# Autodesk Inventor assembly: Gantry2
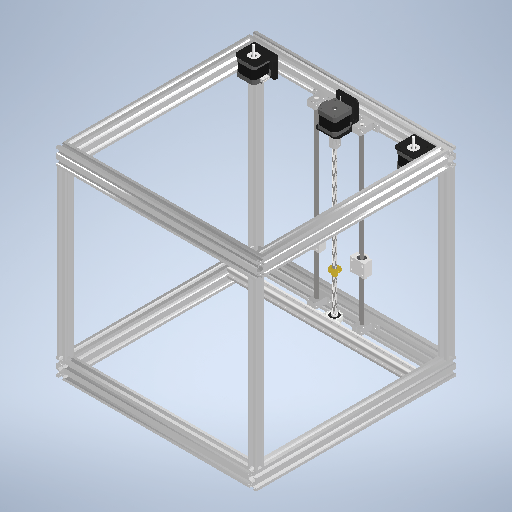
[picture p0: Inventor's stored thumbnail of the model, 512x512]
Saved by Autodesk Inventor 2025.2 (Build 292293000, 293)
## iProperties
Created: 2025-07-13
Part Number: Gantry2
Document SubType Name: Assembly
Designer: Simon
Author: Simon
## Documents named in this file (14)
- C:\Users\Simon\Projects\Hydrogel-3D-Printer\Hardware\Bioprinter Machine Design\Gantry Concept 2\Gantry2.iam
- C:\Users\Simon\Projects\Hydrogel-3D-Printer\Hardware\Bioprinter Machine Design\Gantry Concept 2\2040_AluminimProfile_410.ipt
- C:\Users\Simon\Projects\Hydrogel-3D-Printer\Hardware\Bioprinter Machine Design\Gantry Concept 2\2040_AluminimProfile_450.ipt
- C:\Users\Simon\Projects\Hydrogel-3D-Printer\Hardware\Bioprinter Machine Design\Gantry Concept 2\2020_AluminiumProfile_370.ipt
- C:\Users\Simon\Projects\Hydrogel-3D-Printer\Hardware\Bioprinter Machine Design\PartsFolder\Stepper_17HS4401.ipt
- C:\Users\Simon\Projects\Hydrogel-3D-Printer\Hardware\Bioprinter Machine Design\PartsFolder\bracket nema 17.ipt
- C:\Users\Simon\Projects\Hydrogel-3D-Printer\Hardware\Bioprinter Machine Design\PartsFolder\Pillow Block Bearing 2\KP08_2.iam
- C:\Users\Simon\Projects\Hydrogel-3D-Printer\Hardware\Bioprinter Machine Design\Gantry Concept 2\2020_AluminiumProfile_410.ipt
- C:\Users\Simon\Projects\Hydrogel-3D-Printer\Hardware\Bioprinter Machine Design\Gantry Concept 2\TR8x8-4_LeadScrew_350mm.ipt
- C:\Users\Simon\Projects\Hydrogel-3D-Printer\Hardware\Bioprinter Machine Design\PartsFolder\TR8x8-4_Nut.ipt
- C:\Users\Simon\Projects\Hydrogel-3D-Printer\Hardware\Bioprinter Machine Design\PartsFolder\SK8_LinearShaftSupport.ipt
- C:\Users\Simon\Projects\Hydrogel-3D-Printer\Hardware\Bioprinter Machine Design\PartsFolder\Flexible Coupling 5,8.ipt
- C:\Users\Simon\Projects\Hydrogel-3D-Printer\Hardware\Bioprinter Machine Design\Gantry Concept 2\SteelShaft_404mm.ipt
- C:\Users\Simon\Projects\Hydrogel-3D-Printer\Hardware\Bioprinter Machine Design\PartsFolder\SC8UU\SC8UU.iam
## Components (31 placed, 13 different names)
1. 2040_AluminimProfile_410:1 — Mate:16, Flush:16, Flush:17, Mate:37
2. 2040_AluminimProfile_450:1 — Mate:15, Flush:14, Flush:15, Flush:16, Mate:17, Flush:18, Flush:19, Flush:20, Mate:20, Mate:28, Angle:3, Mate:35, Mate:36, Flush:36, Flush:37
3. 2040_AluminimProfile_410:2 — Mate:6, Mate:7, Flush:3, Angle:2
4. 2040_AluminimProfile_450:2 — Mate:2, Flush:1, Mate:4, Mate:7, Flush:3, Mate:8, Mate:10, Flush:4, Flush:5, Mate:11, Flush:6, Flush:7, Mate:22, Flush:21
5. 2040_AluminimProfile_410:3 — Mate:3, Mate:4, Mate:5, Flush:2
6. 2040_AluminimProfile_450:3 — Mate:1, Flush:1, Mate:5, Flush:2, Mate:9, Mate:12, Mate:13, Flush:8, Flush:9, Flush:10, Flush:11, Mate:29
7. 2040_AluminimProfile_410:4 — Mate:17, Flush:18, Flush:19, Mate:30, Mate:38
8. 2040_AluminimProfile_450:4 — Mate:14, Flush:12, Flush:13, Mate:16, Flush:17
9. 2020_AluminiumProfile_370:1 — Mate:13, Flush:10, Flush:11, Mate:14, Flush:12, Flush:13
10. 2020_AluminiumProfile_370:2 — Mate:12, Flush:8, Flush:9, Mate:15, Flush:14, Flush:15
11. 2020_AluminiumProfile_370:3 — Mate:11, Flush:6, Flush:7
12. 2020_AluminiumProfile_370:4 — Mate:10, Flush:4, Flush:5
13. Stepper_17HS4401:1 — Mate:39, Mate:41, Angle:4
14. Stepper_17HS4401:2 — Mate:40, Mate:42, Angle:5
15. Stepper_17HS4401:3 — Mate:18, Mate:19, Angle:1, Mate:21, Mate:25, Flush:23
16. bracket nema 17:1 — Mate:36, Flush:37, Mate:38, Mate:40, Mate:42, Angle:5
17. bracket nema 17:2 — Mate:18, Mate:19, Angle:1, Mate:20, Flush:20, Mate:31, Mate:32
18. bracket nema 17:3 — Mate:35, Flush:36, Mate:37, Mate:39, Mate:41, Angle:4
19. KP08_2:1 [sub-assembly] — Mate:21, Mate:23, Flush:22, Mate:24, Flush:24
20. 2020_AluminiumProfile_410:1 — Mate:22, Flush:21, Mate:23, Flush:22, Mate:24
21. TR8x8-4_LeadScrew_350mm:1 — Mate:25, Mate:26, Mate:27, Flush:24
22. TR8x8-4_Nut:1 — Mate:26
23. SK8_LinearShaftSupport:1 — Flush:27, Flush:31, Flush:32
24. SK8_LinearShaftSupport:2 — Flush:26, Flush:27, Flush:30, Flush:33
25. SK8_LinearShaftSupport:3 — Flush:25, Mate:28, Flush:28, Flush:32, Mate:31, Mate:33, Flush:34
26. SK8_LinearShaftSupport:4 — Flush:25, Flush:26, Flush:29, Flush:33, Mate:32, Mate:34, Flush:35
27. Flexible Coupling 5,8:1 — Mate:27, Flush:23
28. SteelShaft_404mm:1 — Mate:33, Flush:34, Mate:43
29. SteelShaft_404mm:2 — Mate:34, Flush:35, Mate:44
30. SC8UU:1 [sub-assembly] — Mate:43, Flush:38, Flush:39
31. SC8UU:2 [sub-assembly] — Mate:44, Flush:38, Flush:39
## Relationships (88: Mate 44, Flush 39, Angle 5)
- Mate:1: 2040_AluminimProfile_450:3
- Mate:2: 2040_AluminimProfile_450:2
- Flush:1: 2040_AluminimProfile_450:2 ↔ 2040_AluminimProfile_450:3
- Mate:3: 2040_AluminimProfile_410:3
- Mate:4: 2040_AluminimProfile_450:2 ↔ 2040_AluminimProfile_410:3
- Mate:5: 2040_AluminimProfile_410:3 ↔ 2040_AluminimProfile_450:3
- Flush:2: 2040_AluminimProfile_410:3 ↔ 2040_AluminimProfile_450:3
- Mate:6: 2040_AluminimProfile_410:2
- Mate:7: 2040_AluminimProfile_410:2 ↔ 2040_AluminimProfile_450:2
- Flush:3: 2040_AluminimProfile_410:2 ↔ 2040_AluminimProfile_450:2
- Mate:8: 2040_AluminimProfile_450:2
- Mate:9: 2040_AluminimProfile_450:3
- Mate:10: 2040_AluminimProfile_450:2 ↔ 2020_AluminiumProfile_370:4
- Flush:4: 2040_AluminimProfile_450:2 ↔ 2020_AluminiumProfile_370:4
- Flush:5: 2040_AluminimProfile_450:2 ↔ 2020_AluminiumProfile_370:4
- Mate:11: 2040_AluminimProfile_450:2 ↔ 2020_AluminiumProfile_370:3
- Mate:12: 2040_AluminimProfile_450:3 ↔ 2020_AluminiumProfile_370:2
- Mate:13: 2040_AluminimProfile_450:3 ↔ 2020_AluminiumProfile_370:1
- Flush:6: 2040_AluminimProfile_450:2 ↔ 2020_AluminiumProfile_370:3
- Flush:7: 2040_AluminimProfile_450:2 ↔ 2020_AluminiumProfile_370:3
- Flush:8: 2040_AluminimProfile_450:3 ↔ 2020_AluminiumProfile_370:2
- Flush:9: 2040_AluminimProfile_450:3 ↔ 2020_AluminiumProfile_370:2
- Flush:10: 2040_AluminimProfile_450:3 ↔ 2020_AluminiumProfile_370:1
- Flush:11: 2040_AluminimProfile_450:3 ↔ 2020_AluminiumProfile_370:1
- Mate:14: 2040_AluminimProfile_450:4 ↔ 2020_AluminiumProfile_370:1
- Flush:12: 2040_AluminimProfile_450:4 ↔ 2020_AluminiumProfile_370:1
- Flush:13: 2040_AluminimProfile_450:4 ↔ 2020_AluminiumProfile_370:1
- Mate:15: 2040_AluminimProfile_450:1 ↔ 2020_AluminiumProfile_370:2
- Flush:14: 2040_AluminimProfile_450:1 ↔ 2020_AluminiumProfile_370:2
- Flush:15: 2040_AluminimProfile_450:1 ↔ 2020_AluminiumProfile_370:2
- Mate:16: 2040_AluminimProfile_410:1 ↔ 2040_AluminimProfile_450:4
- Flush:16: 2040_AluminimProfile_410:1 ↔ 2040_AluminimProfile_450:1
- Flush:17: 2040_AluminimProfile_410:1 ↔ 2040_AluminimProfile_450:4
- Mate:17: 2040_AluminimProfile_450:1 ↔ 2040_AluminimProfile_410:4
- Flush:18: 2040_AluminimProfile_450:1 ↔ 2040_AluminimProfile_410:4
- Flush:19: 2040_AluminimProfile_450:1 ↔ 2040_AluminimProfile_410:4
- Mate:18: Stepper_17HS4401:3 ↔ bracket nema 17:2
- Mate:19: Stepper_17HS4401:3 ↔ bracket nema 17:2
- Angle:1 (0 deg): Stepper_17HS4401:3 ↔ bracket nema 17:2
- Mate:20: 2040_AluminimProfile_450:1 ↔ bracket nema 17:2
- Mate:21: Stepper_17HS4401:3 ↔ KP08_2:1
- Flush:20: 2040_AluminimProfile_450:1 ↔ bracket nema 17:2
- Mate:22: 2040_AluminimProfile_450:2 ↔ 2020_AluminiumProfile_410:1
- Flush:21: 2040_AluminimProfile_450:2 ↔ 2020_AluminiumProfile_410:1
- Mate:23: KP08_2:1 ↔ 2020_AluminiumProfile_410:1
- Flush:22: KP08_2:1 ↔ 2020_AluminiumProfile_410:1
- Mate:24: KP08_2:1 ↔ 2020_AluminiumProfile_410:1
- Mate:25: Stepper_17HS4401:3 ↔ TR8x8-4_LeadScrew_350mm:1
- Mate:26: TR8x8-4_LeadScrew_350mm:1 ↔ TR8x8-4_Nut:1
- Mate:27: TR8x8-4_LeadScrew_350mm:1 ↔ Flexible Coupling 5,8:1
- Flush:23 (5 mm): Stepper_17HS4401:3 ↔ Flexible Coupling 5,8:1
- Flush:24: KP08_2:1 ↔ TR8x8-4_LeadScrew_350mm:1
- Flush:25: SK8_LinearShaftSupport:3 ↔ SK8_LinearShaftSupport:4
- Flush:26: SK8_LinearShaftSupport:2 ↔ SK8_LinearShaftSupport:4
- Flush:27: SK8_LinearShaftSupport:1 ↔ SK8_LinearShaftSupport:2
- Mate:28: 2040_AluminimProfile_450:1 ↔ SK8_LinearShaftSupport:3
- Mate:29: 2040_AluminimProfile_450:3
- Angle:2 (0 deg): 2040_AluminimProfile_410:2
- Mate:30: 2040_AluminimProfile_410:4
- Angle:3 (0 deg): 2040_AluminimProfile_450:1
- Flush:28: SK8_LinearShaftSupport:3
- Flush:29: SK8_LinearShaftSupport:4
- Flush:30: SK8_LinearShaftSupport:2
- Flush:31: SK8_LinearShaftSupport:1
- Flush:32: SK8_LinearShaftSupport:1 ↔ SK8_LinearShaftSupport:3
- Flush:33: SK8_LinearShaftSupport:2 ↔ SK8_LinearShaftSupport:4
- Mate:31 (5 mm): bracket nema 17:2 ↔ SK8_LinearShaftSupport:3
- Mate:32 (5 mm): bracket nema 17:2 ↔ SK8_LinearShaftSupport:4
- Mate:33: SK8_LinearShaftSupport:3 ↔ SteelShaft_404mm:1
- Mate:34: SK8_LinearShaftSupport:4 ↔ SteelShaft_404mm:2
- Flush:34: SK8_LinearShaftSupport:3 ↔ SteelShaft_404mm:1
- Flush:35: SK8_LinearShaftSupport:4 ↔ SteelShaft_404mm:2
- Mate:35: 2040_AluminimProfile_450:1 ↔ bracket nema 17:3
- Mate:36: 2040_AluminimProfile_450:1 ↔ bracket nema 17:1
- Flush:36: 2040_AluminimProfile_450:1 ↔ bracket nema 17:3
- Flush:37: 2040_AluminimProfile_450:1 ↔ bracket nema 17:1
- Mate:37: 2040_AluminimProfile_410:1 ↔ bracket nema 17:3
- Mate:38: 2040_AluminimProfile_410:4 ↔ bracket nema 17:1
- Mate:39: Stepper_17HS4401:1 ↔ bracket nema 17:3
- Mate:40: Stepper_17HS4401:2 ↔ bracket nema 17:1
- Mate:41: Stepper_17HS4401:1 ↔ bracket nema 17:3
- Angle:4 (0 deg): Stepper_17HS4401:1 ↔ bracket nema 17:3
- Mate:42: Stepper_17HS4401:2 ↔ bracket nema 17:1
- Angle:5 (0 deg): Stepper_17HS4401:2 ↔ bracket nema 17:1
- Mate:43: SteelShaft_404mm:1 ↔ SC8UU:1
- Mate:44: SteelShaft_404mm:2 ↔ SC8UU:2
- Flush:38: SC8UU:1 ↔ SC8UU:2
- Flush:39: SC8UU:1 ↔ SC8UU:2
